# Autodesk Inventor assembly: Drone Base
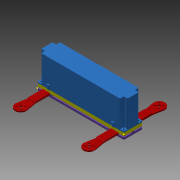
[picture p0: Inventor's stored thumbnail of the model, 180x180]
Saved by Autodesk Inventor 2015 (Build 190159000, 159)
## iProperties
Created: 2016-01-15
Part Number: Drone Base
Document SubType Name: Assembly
Designer: 576994
Author: 576994
## Documents named in this file (10)
- D:\Assignments\EDD\quadparts\Dover's Parts\Drone Base.iam
- D:\Assignments\EDD\quadparts\Dover's Parts\Impact Plate.ipt
- D:\Assignments\EDD\quadparts\Dover's Parts\Arm.ipt
- D:\Assignments\EDD\quadparts\Dover's Parts\Component plate.ipt
- D:\Assignments\EDD\quadparts\Dover's Parts\Arm2.ipt
- D:\Assignments\EDD\quadparts\Camera.ipt
- D:\Assignments\EDD\quadparts\Dover's Parts\BatPlate.ipt
- D:\Assignments\EDD\quadparts\Dover's Parts\Spacer.ipt
- D:\Assignments\EDD\quadparts\Battery.ipt
- D:\Assignments\EDD\quadparts\Dover's Parts\Shell.ipt
## Components (14 placed, 9 different names)
1. Impact Plate:1 — Mate:4, Mate:5, Mate:6, Mate:7, Mate:8, Mate:9, Flush:1, Flush:2, Mate:13, Mate:14, Mate:15, Mate:16, Mate:17, Mate:18, Mate:19
2. Arm:2 — Mate:7, Mate:8, Mate:9
3. Arm:3 — Mate:4, Mate:5, Mate:6
4. Component plate:1 — Flush:1, Flush:2, Mate:13, Flush:5, Flush:7, Flush:8, Mate:25, Mate:26, Flush:9, Mate:28
5. Arm2:2 — Mate:17, Mate:18, Mate:19
6. Arm2:3 — Mate:14, Mate:15, Mate:16
7. Camera:1 — Mate:26
8. BatPlate:1 — Flush:5, Mate:21, Mate:22, Mate:23, Mate:24, Mate:27, Flush:9
9. Spacer:1 — Mate:22, Mate:25
10. Spacer:2 — Mate:24
11. Spacer:3 — Mate:23
12. Spacer:4 — Mate:21
13. Battery:1 — Mate:27
14. Shell:1 — Flush:7, Flush:8, Mate:28
## Relationships (27: Mate 21, Flush 6)
- Mate:4: Impact Plate:1 ↔ Arm:3
- Mate:5: Impact Plate:1 ↔ Arm:3
- Mate:6: Impact Plate:1 ↔ Arm:3
- Mate:7: Impact Plate:1 ↔ Arm:2
- Mate:8: Impact Plate:1 ↔ Arm:2
- Mate:9: Impact Plate:1 ↔ Arm:2
- Flush:1: Impact Plate:1 ↔ Component plate:1
- Flush:2: Impact Plate:1 ↔ Component plate:1
- Mate:13: Impact Plate:1 ↔ Component plate:1
- Mate:14: Impact Plate:1 ↔ Arm2:3
- Mate:15: Impact Plate:1 ↔ Arm2:3
- Mate:16: Impact Plate:1 ↔ Arm2:3
- Mate:17: Impact Plate:1 ↔ Arm2:2
- Mate:18: Impact Plate:1 ↔ Arm2:2
- Mate:19: Impact Plate:1 ↔ Arm2:2
- Flush:5 (3 mm): Component plate:1 ↔ BatPlate:1
- Flush:7: Component plate:1 ↔ Shell:1
- Flush:8: Component plate:1 ↔ Shell:1
- Mate:21: BatPlate:1 ↔ Spacer:4
- Mate:22: BatPlate:1 ↔ Spacer:1
- Mate:23: BatPlate:1 ↔ Spacer:3
- Mate:24: BatPlate:1 ↔ Spacer:2
- Mate:25: Component plate:1 ↔ Spacer:1
- Mate:26: Component plate:1 ↔ Camera:1
- Mate:27: BatPlate:1 ↔ Battery:1
- Flush:9 (17.5 mm): Component plate:1 ↔ BatPlate:1
- Mate:28: Component plate:1 ↔ Shell:1
